# Autodesk Inventor assembly: frame
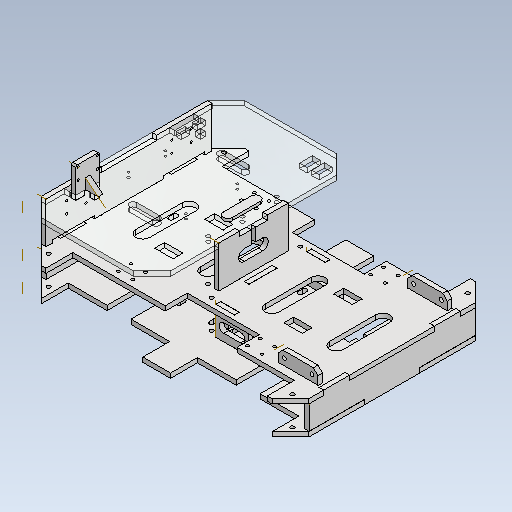
[picture p0: Inventor's stored thumbnail of the model, 512x512]
Saved by Autodesk Inventor 2025 (Build 290162000, 162)
## iProperties
Created: 2025-08-20
Part Number: frame
Document SubType Name: Assembly
Designer: HP
Author: HP
## Documents named in this file (14)
- C:\Users\HP\Documents\GitHub\robotics-dojo-2025\CAD\frame.iam
- C:\Users\HP\Documents\GitHub\robotics-dojo-2025\CAD\floor.ipt
- C:\Users\HP\Documents\GitHub\robotics-dojo-2025\CAD\mid-plate.ipt
- C:\Users\HP\Documents\GitHub\robotics-dojo-2025\CAD\top-plate.ipt
- C:\Users\HP\Documents\GitHub\robotics-dojo-2025\CAD\bed-hinge.ipt
- C:\Users\HP\Documents\GitHub\robotics-dojo-2025\CAD\upper-front-plate-support.ipt
- C:\Users\HP\Documents\GitHub\robotics-dojo-2025\CAD\upper-mid-plate-support.ipt
- C:\Users\HP\Documents\GitHub\robotics-dojo-2025\CAD\lower-mid-plate-support.ipt
- C:\Users\HP\Documents\GitHub\robotics-dojo-2025\CAD\r-support.ipt
- C:\Users\HP\Documents\GitHub\robotics-dojo-2025\CAD\bump-stop.ipt
- C:\Users\HP\Documents\GitHub\robotics-dojo-2025\CAD\lower-front-plate-support.ipt
- C:\Users\HP\Documents\GitHub\robotics-dojo-2025\CAD\lower-back-plate-support.ipt
- C:\Users\HP\Documents\GitHub\robotics-dojo-2025\CAD\camera-bracket-rib.ipt
- C:\Users\HP\Documents\GitHub\robotics-dojo-2025\CAD\camera-bracket.ipt
## Components (15 placed, 13 different names)
1. floor:1 — Mate:1, Flush:1, Flush:2, Flush:5
2. mid-plate:1 — Mate:1, Flush:1, Flush:2, Flush:3, Flush:4, Mate:3, Mate:4, Mate:5, Mate:6, Mate:7, Mate:8, Mate:9, Mate:10, Mate:11, Mate:15, Mate:19, Mate:20, Mate:21, Mate:22, Mate:23, Mate:24, Mate:26, Mate:27, Mate:28, Mate:33, Mate:34, Mate:35, Mate:36, Mate:37
3. top-plate:1 — Flush:3, Flush:4, Mate:12, Mate:13, Mate:14, Mate:25, Mate:32, Mate:38, Mate:40, Mate:41, Mate:42, Mate:43
4. bed-hinge:1 — Mate:6, Mate:7, Mate:8
5. bed-hinge:2 — Mate:3, Mate:4, Mate:5
6. upper-front-plate-support:1 — Mate:9, Mate:10, Mate:11, Mate:32
7. upper-mid-plate-support:1 — Mate:12, Mate:13, Mate:14
8. lower-mid-plate-support:1 — Mate:15, Mate:36, Mate:37
9. r-support:1 — Mate:19, Mate:20, Mate:21
10. r-support:2 — Mate:22, Mate:23, Mate:24
11. bump-stop:1 — Mate:25
12. lower-front-plate-support:1 — Mate:26, Mate:27, Mate:28
13. lower-back-plate-support:1 — Mate:33, Mate:34, Mate:35
14. camera-bracket-rib:1 — Mate:42, Mate:43, Mate:44
15. camera-bracket:1 — Mate:38, Mate:40, Mate:41, Mate:44
## Relationships (41: Mate 36, Flush 5)
- Mate:1 (26 mm): floor:1 ↔ mid-plate:1
- Flush:1: floor:1 ↔ mid-plate:1
- Flush:2: floor:1 ↔ mid-plate:1
- Flush:3: mid-plate:1 ↔ top-plate:1
- Flush:4: mid-plate:1 ↔ top-plate:1
- Mate:3: mid-plate:1 ↔ bed-hinge:2
- Mate:4: mid-plate:1 ↔ bed-hinge:2
- Mate:5: mid-plate:1 ↔ bed-hinge:2
- Mate:6: mid-plate:1 ↔ bed-hinge:1
- Mate:7: mid-plate:1 ↔ bed-hinge:1
- Mate:8: mid-plate:1 ↔ bed-hinge:1
- Mate:9: mid-plate:1 ↔ upper-front-plate-support:1
- Mate:10: mid-plate:1 ↔ upper-front-plate-support:1
- Mate:11: mid-plate:1 ↔ upper-front-plate-support:1
- Mate:12: top-plate:1 ↔ upper-mid-plate-support:1
- Mate:13: top-plate:1 ↔ upper-mid-plate-support:1
- Mate:14: top-plate:1 ↔ upper-mid-plate-support:1
- Mate:15: mid-plate:1 ↔ lower-mid-plate-support:1
- Mate:19: mid-plate:1 ↔ r-support:1
- Mate:20: mid-plate:1 ↔ r-support:1
- Mate:21: mid-plate:1 ↔ r-support:1
- Mate:22: mid-plate:1 ↔ r-support:2
- Mate:23: mid-plate:1 ↔ r-support:2
- Mate:24: mid-plate:1 ↔ r-support:2
- Mate:25: top-plate:1 ↔ bump-stop:1
- Mate:26: mid-plate:1 ↔ lower-front-plate-support:1
- Mate:27: mid-plate:1 ↔ lower-front-plate-support:1
- Mate:28: mid-plate:1 ↔ lower-front-plate-support:1
- Mate:32: top-plate:1 ↔ upper-front-plate-support:1
- Mate:33: mid-plate:1 ↔ lower-back-plate-support:1
- Mate:34: mid-plate:1 ↔ lower-back-plate-support:1
- Mate:35: mid-plate:1 ↔ lower-back-plate-support:1
- Mate:36: mid-plate:1 ↔ lower-mid-plate-support:1
- Mate:37: mid-plate:1 ↔ lower-mid-plate-support:1
- Flush:5: floor:1
- Mate:38: top-plate:1 ↔ camera-bracket:1
- Mate:40: top-plate:1 ↔ camera-bracket:1
- Mate:41: top-plate:1 ↔ camera-bracket:1
- Mate:42: top-plate:1 ↔ camera-bracket-rib:1
- Mate:43: top-plate:1 ↔ camera-bracket-rib:1
- Mate:44: camera-bracket-rib:1 ↔ camera-bracket:1
